# Autodesk Inventor assembly: VersaBlock Assemblyv2
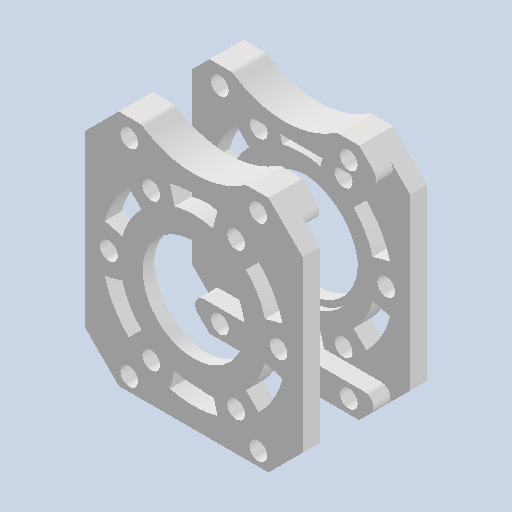
[picture p0: Inventor's stored thumbnail of the model, 512x512]
Saved by Autodesk Inventor 2022 (Build 260153000, 153)
## iProperties
Created: 2020-01-16
Part Number: VersaBlock Assemblyv2
Document SubType Name: Assembly
Designer: aidan
Author: aidan
## Documents named in this file (2)
- C:\Users\tagaz\OneDrive\Documents\T3-Cad\CAD\2022 Parts\VersaBlock Assemblyv2.iam
- C:\Users\tagaz\OneDrive\Documents\T3-Cad\CAD\Versa Chassis Bearing Block.ipt
## Components (2 placed, 1 different names)
1. Versa Chassis Bearing Block:1 — Flush:1, Flush:2, Mate:1
2. Versa Chassis Bearing Block:2 — Flush:1, Flush:2, Mate:1
## Relationships (3: Flush 2, Mate 1)
- Flush:1: Versa Chassis Bearing Block:1 ↔ Versa Chassis Bearing Block:2
- Flush:2: Versa Chassis Bearing Block:1 ↔ Versa Chassis Bearing Block:2
- Mate:1 (25.4 mm): Versa Chassis Bearing Block:1 ↔ Versa Chassis Bearing Block:2
